# Autodesk Inventor assembly: adjustable_double_connector
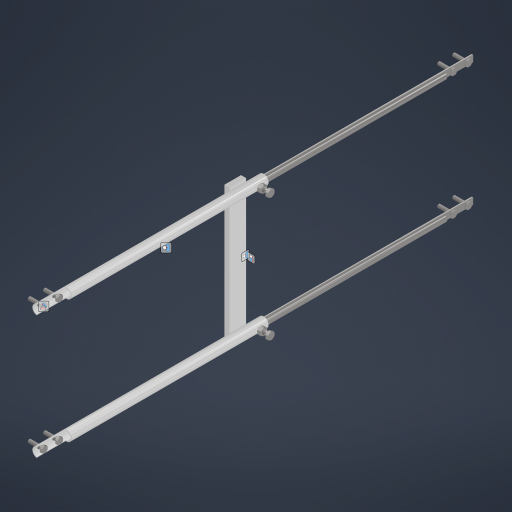
[picture p0: Inventor's stored thumbnail of the model, 512x512]
Saved by Autodesk Inventor 2023 (Build 270158000, 158)
## iProperties
Created: 2022-04-27
Part Number: adjustable_double_connector
Document SubType Name: Assembly
Designer: Norbert Ligas
Author: Norbert Ligas
## Documents named in this file (4)
- C:\Users\norbe\Repozytoria\NormalMapScanner\stand_construction\parts\adjustable_double_connector.iam
- C:\Users\norbe\Repozytoria\NormalMapScanner\stand_construction\parts\adjustable_connector.iam
- C:\Users\norbe\Repozytoria\NormalMapScanner\stand_construction\parts\flat_bar.ipt
- C:\Users\norbe\Repozytoria\NormalMapScanner\stand_construction\parts\adjustable_arm.iam
## Components (3 placed, 2 different names)
1. adjustable_connector:1 [sub-assembly] — Flush:1, Angle:1, Tangent:1, Tangent:2
2. adjustable_connector:2 [sub-assembly] — Angle:2, Tangent:3, Tangent:4, Flush:3
3. flat_bar:2 — Flush:1, Flush:2, Tangent:2, Mate:1, Tangent:4, Flush:3, Mate:3, Mate:4, Mate:5
## Relationships (13: Tangent 4, Mate 4, Flush 3, Angle 2)
- Flush:1 (15 mm): adjustable_connector:1 ↔ flat_bar:2
- Angle:1 (0 deg): adjustable_connector:1
- Tangent:1: adjustable_connector:1
- Flush:2: flat_bar:2
- Tangent:2: adjustable_connector:1 ↔ flat_bar:2
- Angle:2 (0 deg): adjustable_connector:2
- Tangent:3: adjustable_connector:2
- Mate:1: flat_bar:2
- Tangent:4: adjustable_connector:2 ↔ flat_bar:2
- Flush:3 (15 mm): adjustable_connector:2 ↔ flat_bar:2
- Mate:3: flat_bar:2
- Mate:4: flat_bar:2
- Mate:5: flat_bar:2
## Named parameters: pipe_length = 200 mm, iron_angle_to_pipe_edge = 20 mm, flat_bar_length = 160 mm, flat_bar_thickness = 6 mm, flat_bar_width = 20 mm, flat_bar_distance = 15 mm, arm_min_length = 300 mm, arm_max_length = 565 mm
